# Autodesk Inventor assembly: mainflap_side
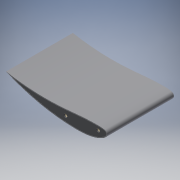
[picture p0: Inventor's stored thumbnail of the model, 180x180]
Saved by Autodesk Inventor 2018.2 (Build 222227000, 227)
## iProperties
Created: 2018-03-05
Part Number: mainflap_side
Material: 一般
Document SubType Name: Assembly
Designer: ku_sk
Author: ku_sk
## Documents named in this file (4)
- D:\ku_sk\ドキュメント\Inventor\Aero\KS-15\Fr.wing\parts\mainflap_side\mainflap_side.iam
- D:\ku_sk\ドキュメント\Inventor\Aero\KS-15\Fr.wing\parts\mainflap_side\plate_ms.ipt
- D:\ku_sk\ドキュメント\Inventor\Aero\KS-15\Fr.wing\parts\mainflap_side\uretan_ms.ipt
- D:\ku_sk\ドキュメント\Inventor\Aero\KS-15\Fr.wing\parts\mainflap_side\GFRP_ms.ipt
## Components (12 placed, 3 different names)
1. plate_ms:1 — フラッシュ:1, メイト:2, メイト:3, メイト:13, メイト:22, メイト:24, メイト:25
2. plate_ms:2 — メイト:1, メイト:2, メイト:3, メイト:4, フラッシュ:2, メイト:5, メイト:14, メイト:29, メイト:30, メイト:31, メイト:32, メイト:33, メイト:34, メイト:35, メイト:36, メイト:37, フラッシュ:11
3. plate_ms:3 — フラッシュ:2, フラッシュ:3, メイト:5, メイト:6, メイト:14, メイト:15, メイト:28
4. plate_ms:4 — フラッシュ:3, メイト:6, メイト:15, フラッシュ:10, メイト:27
5. plate_ms:9 — フラッシュ:9, メイト:12, メイト:21, フラッシュ:10
6. plate_ms:10 — フラッシュ:9, メイト:12, メイト:13, メイト:21, メイト:22, メイト:23, メイト:26
7. uretan_ms:1 — メイト:23, メイト:24, メイト:25, メイト:38
8. uretan_ms:2 — メイト:26, メイト:34, メイト:37
9. uretan_ms:3 — メイト:27, メイト:33, メイト:36, メイト:39
10. uretan_ms:4 — メイト:28, メイト:32, メイト:35
11. uretan_ms:5 — メイト:29, メイト:30, メイト:31
12. GFRP_ms:1 — メイト:38, メイト:39, フラッシュ:11
## Relationships (35: Mate 29, Flush 6)
- フラッシュ:1 [Flush] (-115 mm): plate_ms:1
- メイト:1 [Mate] (-110 mm): plate_ms:2
- メイト:2 [Mate]: plate_ms:1 ↔ plate_ms:2
- メイト:3 [Mate]: plate_ms:1 ↔ plate_ms:2
- メイト:4 [Mate]: plate_ms:2
- フラッシュ:2 [Flush] (-44.2 mm): plate_ms:2 ↔ plate_ms:3
- フラッシュ:3 [Flush] (-44.2 mm): plate_ms:3 ↔ plate_ms:4
- フラッシュ:9 [Flush] (-44.2 mm): plate_ms:9 ↔ plate_ms:10
- メイト:5 [Mate]: plate_ms:2 ↔ plate_ms:3
- メイト:6 [Mate]: plate_ms:3 ↔ plate_ms:4
- メイト:12 [Mate]: plate_ms:9 ↔ plate_ms:10
- メイト:13 [Mate]: plate_ms:1 ↔ plate_ms:10
- メイト:14 [Mate]: plate_ms:2 ↔ plate_ms:3
- メイト:15 [Mate]: plate_ms:3 ↔ plate_ms:4
- メイト:21 [Mate]: plate_ms:9 ↔ plate_ms:10
- メイト:22 [Mate]: plate_ms:1 ↔ plate_ms:10
- フラッシュ:10 [Flush] (-44.2 mm): plate_ms:4 ↔ plate_ms:9
- メイト:23 [Mate]: plate_ms:10 ↔ uretan_ms:1
- メイト:24 [Mate]: plate_ms:1 ↔ uretan_ms:1
- メイト:25 [Mate]: plate_ms:1 ↔ uretan_ms:1
- メイト:26 [Mate]: plate_ms:10 ↔ uretan_ms:2
- メイト:27 [Mate]: plate_ms:4 ↔ uretan_ms:3
- メイト:28 [Mate]: plate_ms:3 ↔ uretan_ms:4
- メイト:29 [Mate]: plate_ms:2 ↔ uretan_ms:5
- メイト:30 [Mate]: plate_ms:2 ↔ uretan_ms:5
- メイト:31 [Mate]: plate_ms:2 ↔ uretan_ms:5
- メイト:32 [Mate]: plate_ms:2 ↔ uretan_ms:4
- メイト:33 [Mate]: plate_ms:2 ↔ uretan_ms:3
- メイト:34 [Mate]: plate_ms:2 ↔ uretan_ms:2
- メイト:35 [Mate]: plate_ms:2 ↔ uretan_ms:4
- メイト:36 [Mate]: plate_ms:2 ↔ uretan_ms:3
- メイト:37 [Mate]: plate_ms:2 ↔ uretan_ms:2
- メイト:38 [Mate]: uretan_ms:1 ↔ GFRP_ms:1
- メイト:39 [Mate]: uretan_ms:3 ↔ GFRP_ms:1
- フラッシュ:11 [Flush]: plate_ms:2 ↔ GFRP_ms:1
